# Autodesk Inventor assembly: M178-PHTM-1000-03
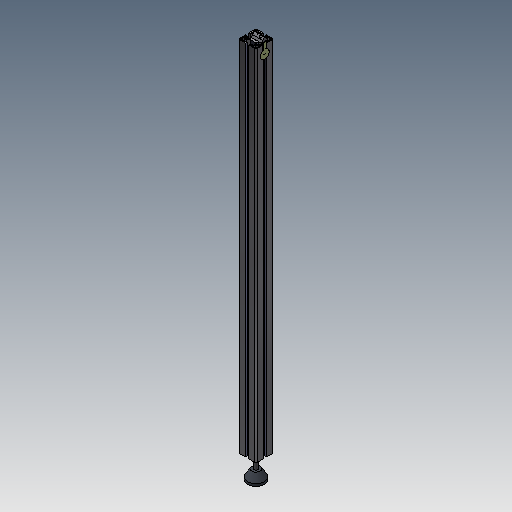
[picture p0: Inventor's stored thumbnail of the model, 512x512]
Saved by Autodesk Inventor 2018.3 (Build 223284000, 284)
## iProperties
Created: 2004-11-18
Part Number: M178-PHTM-1000-03
Document SubType Name: Assembly
Designer: Autodesk, Inc.
Manufacturer: Standard
Standards Organization: Custom
Description: PHANTOM, TABLE, LEGS
Mass: 1519.64 g
Surface Area: 3943.48 cm^2
Volume: 557.12 cm^3
Density: 2.72766 g/cm^3
CAGE: 1LJX3
Dept. ID: Product Design
Description #2: ---
Finish #1: ---
Finish #2: ---
Material ID: ---
Project Number: ---
Author: Autodesk, Inc.
## Documents named in this file (8)
- C:\AVAInvAPI\Workspace\Test Station\Components\M178-1000_Leg_Phantom.iam
- C:\AVAInvAPI\Workspace\Test Station\Components\21-009.ipt
- C:\AVAInvAPI\Workspace\Test Station\Components\M178-1004.ipt
- C:\AVAInvAPI\Workspace\Test Station\Components\20-004.iam
- C:\AVAInvAPI\Workspace\Test Station\Components\24-706-8.ipt
- C:\Users\kelleyb.ADS\Desktop\Samples MIGRATED 2009 224 RTM_1\Standard Parts\Test Station Content\Misc Hardware\21-0xx Knuckle Foot.ipt
- C:\Users\kelleyb.ADS\Desktop\Samples MIGRATED 2009 224 RTM_1\Standard Parts\Test Station Content\Fastners\24-7X6 Hexagon Nuts.ipt
- C:\Users\kelleyb.ADS\Desktop\Samples MIGRATED 2009 224 RTM_1\Standard Parts\Test Station Content\Extrusions\40 Series Profiles.ipt
## Components (4 placed, 4 different names)
1. 21-009:1
2. 24-706-8:1
3. M178-1004:1
4. 20-004:1 [sub-assembly]
## Relationships (4: Insert 2, Mate 1, Angle 1)
- [Insert] (20 mm): 21-009:1 ↔ 24-706-8:1
- [Mate]: 21-009:1 ↔ M178-1004:1
- [Insert]: M178-1004:1 ↔ 20-004:1
- [Angle] (0 deg): M178-1004:1 ↔ 20-004:1
